# Autodesk Inventor assembly: DarkPoolFacility
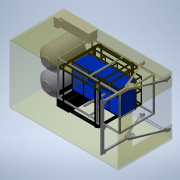
[picture p0: Inventor's stored thumbnail of the model, 180x180]
Saved by Autodesk Inventor 2022 (Build 260153000, 153)
## iProperties
Created: 2021-05-11
Part Number: DarkPoolFacility
Document SubType Name: Assembly
Designer: jamieson-bl
Author: jamieson-bl
## Documents named in this file (12)
- \\Mac\Home\Desktop\WinnipegPMTTestFacility\DarkPoolFacility.iam
- \\Mac\Home\Desktop\WinnipegPMTTestFacility\iManikins\iMan\iMan.iam
- \\Mac\Home\Desktop\WinnipegPMTTestFacility\iManikins\iMandy\iMandy.iam
- \\Mac\Home\Desktop\WinnipegPMTTestFacility\Field Compensation Coils.iam
- \\Mac\Home\Desktop\WinnipegPMTTestFacility\ElectronicsRack.ipt
- \\Mac\Home\Desktop\WinnipegPMTTestFacility\CustomAquariumsStand.ipt
- \\Mac\Home\Desktop\WinnipegPMTTestFacility\CustomAquariumsTank.ipt
- \\Mac\Home\Desktop\WinnipegPMTTestFacility\gantry design\6060gantry.iam
- \\Mac\Home\Desktop\WinnipegPMTTestFacility\Room_0RC039.ipt
- \\Mac\Home\Desktop\WinnipegPMTTestFacility\DuraCast_V325Gallon.ipt
- \\Mac\Home\Desktop\WinnipegPMTTestFacility\SumpAssembly.iam
- \\Mac\Home\Desktop\WinnipegPMTTestFacility\3775T610_MOBILE EASY-STORE ADJUSTABLE ALUMINUM CRANE McMaster.ipt
## Components (12 placed, 11 different names)
1. iMan:1 [sub-assembly]
2. iMandy:1 [sub-assembly]
3. Field Compensation Coils:1 [sub-assembly] — Mate:5, Mate:6, Mate:7
4. ElectronicsRack:1 — Mate:13
5. CustomAquariumsStand:1 — Mate:4, Flush:1, Flush:2, Mate:5, Mate:6, Flush:3, Mate:9, Mate:10
6. CustomAquariumsTank:1 — Mate:4, Flush:1, Flush:2, Mate:7, Mate:8
7. 6060gantry:1 [sub-assembly] — Flush:3, Mate:8, Mate:9
8. Room_0RC039:1 — Mate:10, Mate:13, Mate:15, Mate:16, Mate:17, Mate:18
9. DuraCast_V325Gallon:1 — Mate:15
10. DuraCast_V325Gallon:3 — Mate:16
11. SumpAssembly:1 [sub-assembly] — Mate:17
12. 3775T610_MOBILE EASY-STORE ADJUSTABLE ALUMINUM CRANE McMaster:1 — Mate:18
## Relationships (15: Mate 12, Flush 3)
- Mate:4: CustomAquariumsStand:1 ↔ CustomAquariumsTank:1
- Flush:1: CustomAquariumsStand:1 ↔ CustomAquariumsTank:1
- Flush:2: CustomAquariumsStand:1 ↔ CustomAquariumsTank:1
- Mate:5: Field Compensation Coils:1 ↔ CustomAquariumsStand:1
- Mate:6: Field Compensation Coils:1 ↔ CustomAquariumsStand:1
- Mate:7: Field Compensation Coils:1 ↔ CustomAquariumsTank:1
- Flush:3: CustomAquariumsStand:1 ↔ 6060gantry:1
- Mate:8: CustomAquariumsTank:1 ↔ 6060gantry:1
- Mate:9: CustomAquariumsStand:1 ↔ 6060gantry:1
- Mate:10: CustomAquariumsStand:1 ↔ Room_0RC039:1
- Mate:13: ElectronicsRack:1 ↔ Room_0RC039:1
- Mate:15: Room_0RC039:1 ↔ DuraCast_V325Gallon:1
- Mate:16: Room_0RC039:1 ↔ DuraCast_V325Gallon:3
- Mate:17: Room_0RC039:1 ↔ SumpAssembly:1
- Mate:18 (185.42 mm): Room_0RC039:1 ↔ 3775T610_MOBILE EASY-STORE ADJUSTABLE ALUMINUM CRANE McMaster:1
